# Autodesk Inventor assembly: center piece
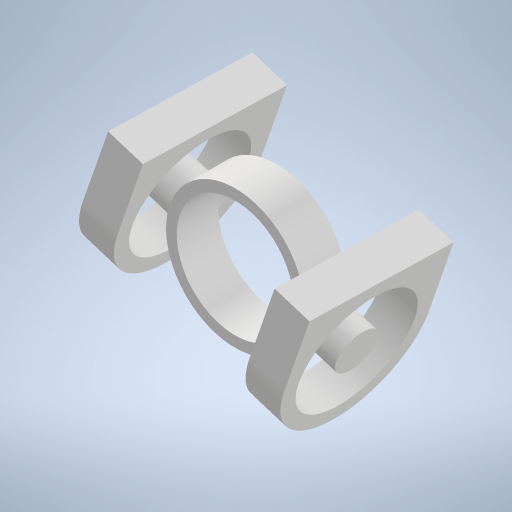
[picture p0: Inventor's stored thumbnail of the model, 512x512]
Saved by Autodesk Inventor 2024 (Build 280153000, 153)
## iProperties
Created: 2024-04-03
Part Number: center piece
Document SubType Name: Assembly
Designer: compu
Author: compu
## Documents named in this file (3)
- C:\Users\compu\Documents\1Juan\1Facultad\9 Semestre\E1225 Taller de Sistemas Digitales\Parts\center piece\center piece.iam
- C:\Users\compu\Documents\1Juan\1Facultad\9 Semestre\E1225 Taller de Sistemas Digitales\Parts\center piece\anillo central.ipt
- C:\Users\compu\Documents\1Juan\1Facultad\9 Semestre\E1225 Taller de Sistemas Digitales\Parts\center piece\laterales.ipt
## Components (3 placed, 2 different names)
1. anillo central:1 — Mate:1, Flush:1, Insert:1, Insert:2
2. laterales:1 — Insert:1, Flush:2
3. laterales:2 — Insert:2, Flush:2
## Relationships (5: Flush 2, Insert 2, Mate 1)
- Mate:1: anillo central:1
- Flush:1: anillo central:1
- Insert:1: anillo central:1 ↔ laterales:1
- Insert:2: anillo central:1 ↔ laterales:2
- Flush:2: laterales:1 ↔ laterales:2
